# Autodesk Inventor assembly: Planktoscope_Mini_Peristalticpump_new
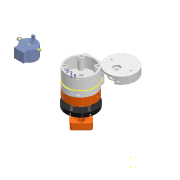
[picture p0: Inventor's stored thumbnail of the model, 180x180]
Saved by Autodesk Inventor 2022.5 (Build 265521000, 521)
## iProperties
Created: 2022-11-30
Part Number: Planktoscope_Mini_Peristalticpump_new
Document SubType Name: Assembly
Designer: diederichbenedict
Author: diederichbenedict
## Documents named in this file (9)
- C:\Users\diederichbenedict\Dropbox\Dokumente\Promotion\PROJECTS\Matchboxscope\INVENTOR\RELEASE\PlanktoscopeMini\Workspace\Planktoscope_Mini_Peristalticpump_new.iam
- C:\Users\diederichbenedict\Dropbox\Dokumente\Promotion\PROJECTS\Matchboxscope\INVENTOR\RELEASE\PlanktoscopeMini\Workspace\00_Stepper_Motor_28BYJ-48.ipt
- C:\Users\diederichbenedict\Dropbox\Dokumente\Promotion\PROJECTS\Matchboxscope\INVENTOR\RELEASE\PlanktoscopeMini\Workspace\Matchboxscope_bottom_v0.ipt
- C:\Users\diederichbenedict\Dropbox\Dokumente\Promotion\PROJECTS\openUC2-CAD\INVENTOR\Pump_Base_Motor_tubeholder_new_.ipt
- C:\Users\diederichbenedict\Dropbox\Dokumente\Promotion\PROJECTS\Matchboxscope\INVENTOR\RELEASE\PlanktoscopeMini\Workspace\Pump_Base_Motor_tubeholder_new.ipt
- C:\Users\diederichbenedict\Dropbox\Dokumente\Promotion\PROJECTS\Matchboxscope\INVENTOR\RELEASE\PlanktoscopeMini\Workspace\Pump_Rotatio_new.ipt
- C:\Users\diederichbenedict\Dropbox\Dokumente\Promotion\PROJECTS\Matchboxscope\INVENTOR\RELEASE\PlanktoscopeMini\Workspace\Pump_Base_Motor_new.ipt
- C:\Users\diederichbenedict\Dropbox\Dokumente\Promotion\PROJECTS\Matchboxscope\INVENTOR\RELEASE\PlanktoscopeMini\Workspace\00_Bearing_4x13.5.ipt
- C:\Users\diederichbenedict\Dropbox\Dokumente\Promotion\PROJECTS\Matchboxscope\INVENTOR\RELEASE\ESPressoscope_XIAO\Workspace\Assembly_Matchboxscope_injectionmolded_xiao.iam
## Components (12 placed, 8 different names)
1. 00_Stepper_Motor_28BYJ-48:1 — Passend:2, Passend:3
2. Matchboxscope_bottom_v0:1 — Passend:2, Passend:3
3. Pump_Base_Motor_tubeholder_new:1 — Einfügen:1, Einfügen:2, Einfügen:8
4. Pump_Base_Motor_tubeholder_new_:1 — Einfügen:7
5. Pump_Rotatio_new:1 — Einfügen:2, Einfügen:3, Einfügen:4
6. Pump_Base_Motor_new:1 — Einfügen:1
7. 00_Bearing_4x13.5:1 — Einfügen:3
8. 00_Bearing_4x13.5:2 — Einfügen:4
9. Pump_Rotatio_new:2 — Einfügen:7
10. 00_Bearing_4x13.5:3
11. 00_Bearing_4x13.5:4
12. Assembly_Matchboxscope_injectionmolded_xiao:1 [sub-assembly] — Einfügen:8
## Relationships (10: Insert 8, Mate 2)
- Passend:2 [Mate]: 00_Stepper_Motor_28BYJ-48:1 ↔ Matchboxscope_bottom_v0:1
- Passend:3 [Mate] (20 mm): 00_Stepper_Motor_28BYJ-48:1 ↔ Matchboxscope_bottom_v0:1
- Einfügen:1 [Insert]: Pump_Base_Motor_tubeholder_new:1 ↔ Pump_Base_Motor_new:1
- Einfügen:2 [Insert]: Pump_Base_Motor_tubeholder_new:1 ↔ Pump_Rotatio_new:1
- Einfügen:3 [Insert]: Pump_Rotatio_new:1 ↔ 00_Bearing_4x13.5:1
- Einfügen:4 [Insert]: Pump_Rotatio_new:1 ↔ 00_Bearing_4x13.5:2
- [Insert]: Pump_Rotatio_new:2 ↔ 00_Bearing_4x13.5:3
- [Insert]: Pump_Rotatio_new:2 ↔ 00_Bearing_4x13.5:4
- Einfügen:7 [Insert]: Pump_Base_Motor_tubeholder_new_:1 ↔ Pump_Rotatio_new:2
- Einfügen:8 [Insert]: Pump_Base_Motor_tubeholder_new:1 ↔ Assembly_Matchboxscope_injectionmolded_xiao:1
## Named parameters: d22_d20 = 0 mm, d23_d21 = 0 mm
